# Autodesk Inventor assembly: drop_center_wheel
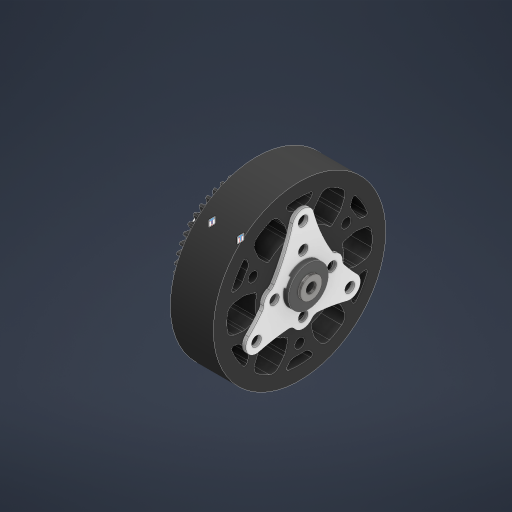
[picture p0: Inventor's stored thumbnail of the model, 512x512]
Saved by Autodesk Inventor 2024 (Build 280153000, 153)
## iProperties
Created: 2023-10-29
Part Number: drop_center_wheel
Document SubType Name: Assembly
Designer: avere
Author: avere
## Documents named in this file (12)
- C:\Users\avere\Documents\rbp_cad\zoomba_v0.1\chassis\drivebay\drop_center_wheel.iam
- C:\Users\avere\Documents\rbp_cad\VEX-CAD-Inventor-1.41\Motion\Wheels\Flex Wheels\3.000 Flex Wheel.ipt
- C:\Users\avere\Documents\rbp_cad\VEX-CAD-Inventor-1.41\Motion\Wheels\Flex Wheels\3.000 Flex Wheel\3.000 60A .750.ipt
- C:\Users\avere\Documents\rbp_cad\zoomba_v0.1\chassis\drivebay\custom_parts\drop_center_hub.ipt
- C:\Users\avere\Documents\rbp_cad\VEX-CAD-Inventor-1.41\Motion\Wheels\Flex Wheels\VersaHex Adapters .250.ipt
- C:\Users\avere\Documents\rbp_cad\VEX-CAD-Inventor-1.41\Motion\Spacers\Spacer Nylon .375 OD.ipt
- C:\Users\avere\Documents\rbp_cad\zoomba_v0.1\chassis\drivebay\custom_parts\washer_thin.ipt
- C:\Users\avere\Documents\rbp_cad\zoomba_v0.1\chassis\drivebay\custom_parts\ls_48t_flat.ipt
- C:\Users\avere\Documents\rbp_cad\VEX-CAD-Inventor-1.41\Motion\Spacers\Washer Steel\SWasher .375 OD x .031250.ipt
- C:\Users\avere\Documents\rbp_cad\VEX-CAD-Inventor-1.41\Motion\Spacers\Washer Steel.ipt
- C:\Users\avere\Documents\rbp_cad\VEX-CAD-Inventor-1.41\Motion\Spacers\Washer Steel\SWasher .375 OD x .015625.ipt
- C:\Users\avere\Documents\rbp_cad\VEX-CAD-Inventor-1.41\Motion\Spacers\Spacer Nylon .375 OD\NSpacer .375 OD x .500.ipt
## Components (10 placed, 8 different names)
1. drop_center_hub:1 — Mate:2, Insert:9
2. 3.000 60A .750:1 — Mate:2, Insert:3, Mate:3, Insert:4, Insert:8, Insert:9
3. drop_center_hub:2 — Insert:3, Mate:3
4. VersaHex Adapters .250:1 — Insert:4, Insert:13
5. washer_thin:1 — Insert:15
6. VersaHex Adapters .250:2 — Insert:8, Insert:10
7. ls_48t_flat:1 — Insert:10, Insert:14
8. SWasher .375 OD x .031250:1 — Insert:12, Insert:13
9. SWasher .375 OD x .015625:2 — Insert:12
10. NSpacer .375 OD x .500:1 — Insert:14, Insert:15
## Relationships (11: Insert 9, Mate 2)
- Mate:2: drop_center_hub:1 ↔ 3.000 60A .750:1
- Insert:3: 3.000 60A .750:1 ↔ drop_center_hub:2
- Mate:3: 3.000 60A .750:1 ↔ drop_center_hub:2
- Insert:4 (1.5875 mm): 3.000 60A .750:1 ↔ VersaHex Adapters .250:1
- Insert:8 (1.5875 mm): 3.000 60A .750:1 ↔ VersaHex Adapters .250:2
- Insert:9: drop_center_hub:1 ↔ 3.000 60A .750:1
- Insert:10 (-3.175 mm): VersaHex Adapters .250:2 ↔ ls_48t_flat:1
- Insert:12: SWasher .375 OD x .031250:1 ↔ SWasher .375 OD x .015625:2
- Insert:13: VersaHex Adapters .250:1 ↔ SWasher .375 OD x .031250:1
- Insert:14 (-3.175 mm): ls_48t_flat:1 ↔ NSpacer .375 OD x .500:1
- Insert:15: washer_thin:1 ↔ NSpacer .375 OD x .500:1
